# Autodesk Inventor assembly: ABD_Version_0.1_leftleg
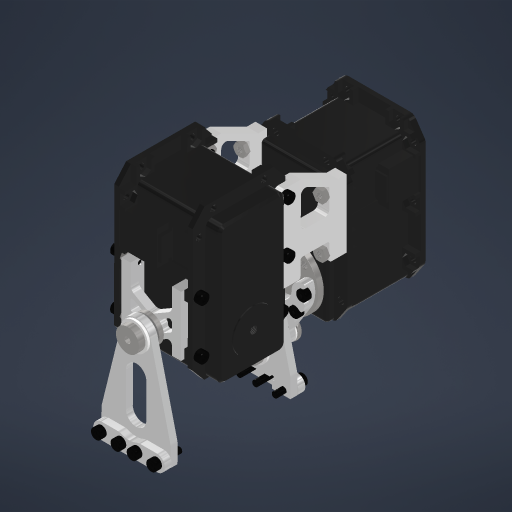
[picture p0: Inventor's stored thumbnail of the model, 512x512]
Saved by Autodesk Inventor 2024.3 (Build 283343000, 343)
## iProperties
Created: 2024-01-23
Part Number: ABD_Version_0.1_leftleg
Document SubType Name: Assembly
Designer: ASUS
Mass: 357.136 g
Surface Area: 604.848 cm^2
Volume: 181.423 cm^3
Density: 1.96853 g/cm^3
Author: ASUS
## Documents named in this file (18)
- C:\Users\ASUS\Desktop\test\v4_Frame_2025\ABD_V4_Right_OP.iam
- C:\Users\ASUS\Desktop\test\v4_Frame_2025\ABD_Slider_Set_v4.iam
- C:\Users\ASUS\Desktop\test\v4_Frame_2025\Roll_Fixation_Frame_Back.ipt
- C:\Users\ASUS\Desktop\test\v4_Frame_2025\hip joint fix washer.ipt
- C:\Users\ASUS\Desktop\test\Screw_Set\hip_joint_fix_washer_10mm_Set.iam
- C:\Users\ASUS\Desktop\test\v4_Frame_2025\Front_Frame_Fixer_v2.iam
- C:\Users\ASUS\Desktop\test\ROBOTIS(Inventor 2024 ver.)\DXL\MX-64T.ipt
- C:\Users\ASUS\Desktop\test\v2_Frame\MISUMI\DBSY4-5-8.ipt
- C:\Users\ASUS\Desktop\test\v4_Frame_2025\Dynamixel Vertical fixation.ipt
- C:\Users\ASUS\Desktop\test\v4_Frame_2025\Dynamixel Vertical fixation_MIR.ipt
- C:\Users\ASUS\Desktop\test\v1_Frame\MISUMI\SLBNR2_5.ipt
- C:\Users\ASUS\Desktop\test\Screw_Set\Roll_Fixation_Frame_8mm_Set.iam
- C:\Users\ASUS\Desktop\test\v4_Frame_2025\Roll_Fixation_R.ipt
- C:\Users\ASUS\Desktop\test\v4_Frame_2025\Roll_Fixation_L.ipt
- C:\Users\ASUS\Desktop\test\ROBOTIS(Inventor 2024 ver.)\DXL\MX-106T.ipt
- C:\Users\ASUS\Desktop\test\Screw_Set\Roll_Fixation_Frame_8mm_Set_Backside.iam
- C:\Users\ASUS\Desktop\test\v4_Frame\MISUMI\DBGS4-5-8.ipt
- C:\Users\ASUS\Desktop\test\v4_Frame_2025\Crank_Fixation.iam
## Components (24 placed, 17 different names)
1. hip joint fix washer:1 — 삽입:64
2. hip joint fix washer:2 — 삽입:47, 메이트:29
3. hip_joint_fix_washer_10mm_Set:1 [sub-assembly] — 메이트:39
4. hip_joint_fix_washer_10mm_Set:2 [sub-assembly] — 메이트:29
5. Front_Frame_Fixer_v2:1 [sub-assembly] — 삽입:63, 삽입:78, 삽입:81
6. DBSY4-5-8:1 — 삽입:81
7. MX-64T:1 — 삽입:43, 메이트:35, 메이트:36, 각도:14, 각도:15, 삽입:89, 삽입:90, 메이트:61
8. ABD_Slider_Set_v4:2 [sub-assembly] — 삽입:43, 삽입:88
9. Roll_Fixation_Frame_Back:3 — 삽입:47, 메이트:58, 메이트:59, 각도:15, 메이트:60
10. Front_Frame_Fixer_v2:2 [sub-assembly] — 삽입:77, 메이트:58, 메이트:59, 삽입:87
11. Dynamixel Vertical fixation:2 — 메이트:35, 삽입:89
12. Dynamixel Vertical fixation_MIR:2 — 메이트:36, 메이트:54, 메이트:55, 메이트:56, 삽입:90, 메이트:61
13. SLBNR2_5:5
14. SLBNR2_5:6
15. SLBNR2_5:7
16. SLBNR2_5:8
17. Roll_Fixation_Frame_Back:4 — 삽입:63, 메이트:39, 삽입:64
18. Roll_Fixation_R:1 — 삽입:78
19. Roll_Fixation_L:1 — 삽입:77
20. MX-106T:1 — 각도:14, 삽입:79, 메이트:52, 삽입:80, 메이트:53, 메이트:56
21. Roll_Fixation_Frame_8mm_Set:1 [sub-assembly] — 삽입:80, 메이트:53
22. Roll_Fixation_Frame_8mm_Set_Backside:1 [sub-assembly] — 삽입:79, 메이트:52, 메이트:54, 메이트:55
23. DBGS4-5-8:1 — 삽입:87
24. Crank_Fixation:1 [sub-assembly] — 삽입:88, 메이트:60
## Relationships (48: Mate 22, Insert 19, Angle 6, Flush 1)
- [Insert]: hip joint fix washer:1 ↔ hip_joint_fix_washer_10mm_Set:1
- [Mate]: hip joint fix washer:1 ↔ hip_joint_fix_washer_10mm_Set:1
- [Insert]: hip joint fix washer:2 ↔ hip_joint_fix_washer_10mm_Set:2
- [Mate]: hip joint fix washer:2 ↔ hip_joint_fix_washer_10mm_Set:2
- [Mate]: hip_joint_fix_washer_10mm_Set:1 ↔ hip_joint_fix_washer_10mm_Set:2
- [Mate]: hip_joint_fix_washer_10mm_Set:1 ↔ hip_joint_fix_washer_10mm_Set:2
- 삽입:43 [Insert] (0.5 mm): MX-64T:1 ↔ ABD_Slider_Set_v4:2
- 삽입:47 [Insert]: hip joint fix washer:2 ↔ Roll_Fixation_Frame_Back:3
- 메이트:29 [Mate]: hip joint fix washer:2 ↔ hip_joint_fix_washer_10mm_Set:2
- [Insert]: Dynamixel Vertical fixation:2 ↔ SLBNR2_5:5
- [Insert]: Dynamixel Vertical fixation:2 ↔ SLBNR2_5:6
- [Insert]: Dynamixel Vertical fixation_MIR:2 ↔ SLBNR2_5:8
- [Insert]: Dynamixel Vertical fixation_MIR:2 ↔ SLBNR2_5:7
- [Angle] (0 deg): Dynamixel Vertical fixation_MIR:2 ↔ SLBNR2_5:7
- [Angle] (0 deg): Dynamixel Vertical fixation_MIR:2 ↔ SLBNR2_5:8
- [Angle] (0 deg): Dynamixel Vertical fixation:2 ↔ SLBNR2_5:5
- [Angle] (0 deg): Dynamixel Vertical fixation:2 ↔ SLBNR2_5:6
- 메이트:35 [Mate]: MX-64T:1 ↔ Dynamixel Vertical fixation:2
- 메이트:36 [Mate]: MX-64T:1 ↔ Dynamixel Vertical fixation_MIR:2
- 삽입:63 [Insert]: Front_Frame_Fixer_v2:1 ↔ Roll_Fixation_Frame_Back:4
- 메이트:39 [Mate]: hip_joint_fix_washer_10mm_Set:1 ↔ Roll_Fixation_Frame_Back:4
- 삽입:64 [Insert]: hip joint fix washer:1 ↔ Roll_Fixation_Frame_Back:4
- [Flush]: Roll_Fixation_R:1 ↔ Roll_Fixation_L:1
- [Mate] (0.05 mm): Roll_Fixation_R:1 ↔ MX-106T:1
- [Mate] (0.05 mm): Roll_Fixation_L:1 ↔ MX-106T:1
- [Mate]: Roll_Fixation_L:1 ↔ MX-106T:1
- [Mate]: Roll_Fixation_L:1 ↔ MX-106T:1
- [Mate]: Roll_Fixation_R:1 ↔ MX-106T:1
- 삽입:77 [Insert]: Front_Frame_Fixer_v2:2 ↔ Roll_Fixation_L:1
- 각도:14 [Angle] (0 deg): MX-64T:1 ↔ MX-106T:1
- 삽입:78 [Insert]: Front_Frame_Fixer_v2:1 ↔ Roll_Fixation_R:1
- 삽입:79 [Insert]: MX-106T:1 ↔ Roll_Fixation_Frame_8mm_Set_Backside:1
- 메이트:52 [Mate]: MX-106T:1 ↔ Roll_Fixation_Frame_8mm_Set_Backside:1
- 삽입:80 [Insert]: MX-106T:1 ↔ Roll_Fixation_Frame_8mm_Set:1
- 메이트:53 [Mate]: MX-106T:1 ↔ Roll_Fixation_Frame_8mm_Set:1
- 메이트:54 [Mate]: Dynamixel Vertical fixation_MIR:2 ↔ Roll_Fixation_Frame_8mm_Set_Backside:1
- 메이트:55 [Mate]: Dynamixel Vertical fixation_MIR:2 ↔ Roll_Fixation_Frame_8mm_Set_Backside:1
- 메이트:56 [Mate] (0.05 mm): Dynamixel Vertical fixation_MIR:2 ↔ MX-106T:1
- 삽입:81 [Insert]: Front_Frame_Fixer_v2:1 ↔ DBSY4-5-8:1
- 메이트:58 [Mate]: Roll_Fixation_Frame_Back:3 ↔ Front_Frame_Fixer_v2:2
- 메이트:59 [Mate]: Roll_Fixation_Frame_Back:3 ↔ Front_Frame_Fixer_v2:2
- 삽입:87 [Insert]: Front_Frame_Fixer_v2:2 ↔ DBGS4-5-8:1
- 각도:15 [Angle] (0 deg): MX-64T:1 ↔ Roll_Fixation_Frame_Back:3
- 삽입:88 [Insert]: ABD_Slider_Set_v4:2 ↔ Crank_Fixation:1
- 메이트:60 [Mate]: Roll_Fixation_Frame_Back:3 ↔ Crank_Fixation:1
- 삽입:89 [Insert]: MX-64T:1 ↔ Dynamixel Vertical fixation:2
- 삽입:90 [Insert]: MX-64T:1 ↔ Dynamixel Vertical fixation_MIR:2
- 메이트:61 [Mate]: MX-64T:1 ↔ Dynamixel Vertical fixation_MIR:2
## Named parameters: d1061_d1053 = 0 mm, d1062_d1054 = 0 mm, d1063_d1055 = 0 mm, d1064_d1056 = 0 mm, d1065_d1057 = 0 deg, d1066_d1058 = 0 deg, d1067_d1059 = 0 deg, d1068_d1060 = 0 deg, d1081_d18 = 0.05 mm
